# Autodesk Inventor assembly: ASM1001-001-005-320 - Controller Flash
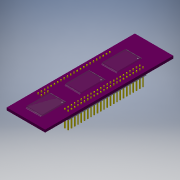
[picture p0: Inventor's stored thumbnail of the model, 180x180]
Saved by Autodesk Inventor 2019 (Build 230136000, 136)
## iProperties
Created: 2019-07-16
Part Number: ASM1001-001-005-320 - Controller Flash
Document SubType Name: Assembly
Designer: james
Author: james
## Documents named in this file (6)
- F:\JimsDesign\P1001-16bit-CPU\P1001-001 - 16bit CPU\P1001-001-005-320 - Controller Flash\ASM1001-001-005-320 - Controller Flash.iam
- F:\JimsDesign\P1001-16bit-CPU\P1001-001 - 16bit CPU\P1001-001-005-320 - Controller Flash\PRT1001-001-005-320 - Controller Flash.ipt
- F:\JimsDesign\P1001-16bit-CPU\P1001-001 - 16bit CPU\P1001-001-210 - CAD Library\UL_SST39VF1602704IEKE\2019-07-17_03-10-51\STEP\TSOP48_EKE_SST.ipt
- F:\JimsDesign\P1001-16bit-CPU\P1001-001 - 16bit CPU\P1001-001-210 - CAD Library\2X24Pins.iam
- F:\JimsDesign\P1001-16bit-CPU\P1001-001 - 16bit CPU\P1001-001-210 - CAD Library\1x20Pins.iam
- F:\JimsDesign\P1001-16bit-CPU\P1001-001 - 16bit CPU\P1001-001-210 - CAD Library\2x3pins.iam
## Components (7 placed, 5 different names)
1. PRT1001-001-005-320 - Controller Flash:1 — Mate:1, Mate:2, Mate:3, Mate:4, Mate:6, Flush:5, Flush:6, Mate:7, Flush:7, Flush:8
2. TSOP48_EKE_SST:1 — Mate:3, Flush:2
3. TSOP48_EKE_SST:2 — Mate:2, Flush:1, Flush:2
4. TSOP48_EKE_SST:3 — Mate:1, Mate:4, Flush:1
5. 2X24Pins:1 [sub-assembly] — Mate:7, Flush:7, Flush:8
6. 1x20Pins:1 [sub-assembly] — Mate:5, Flush:3, Flush:4, Mate:6, Flush:5
7. 2x3pins:1 [sub-assembly] — Mate:5, Flush:3, Flush:4, Flush:6
## Relationships (15: Flush 8, Mate 7)
- Mate:1: PRT1001-001-005-320 - Controller Flash:1 ↔ TSOP48_EKE_SST:3
- Mate:2: PRT1001-001-005-320 - Controller Flash:1 ↔ TSOP48_EKE_SST:2
- Mate:3: PRT1001-001-005-320 - Controller Flash:1 ↔ TSOP48_EKE_SST:1
- Mate:4 (10 mm): PRT1001-001-005-320 - Controller Flash:1 ↔ TSOP48_EKE_SST:3
- Flush:1: TSOP48_EKE_SST:2 ↔ TSOP48_EKE_SST:3
- Flush:2: TSOP48_EKE_SST:1 ↔ TSOP48_EKE_SST:2
- Mate:5: 1x20Pins:1 ↔ 2x3pins:1
- Flush:3: 1x20Pins:1 ↔ 2x3pins:1
- Flush:4: 1x20Pins:1 ↔ 2x3pins:1
- Mate:6: PRT1001-001-005-320 - Controller Flash:1 ↔ 1x20Pins:1
- Flush:5 (2 mm): PRT1001-001-005-320 - Controller Flash:1 ↔ 1x20Pins:1
- Flush:6 (20 mm): PRT1001-001-005-320 - Controller Flash:1 ↔ 2x3pins:1
- Mate:7: PRT1001-001-005-320 - Controller Flash:1 ↔ 2X24Pins:1
- Flush:7 (20 mm): PRT1001-001-005-320 - Controller Flash:1 ↔ 2X24Pins:1
- Flush:8 (2 mm): PRT1001-001-005-320 - Controller Flash:1 ↔ 2X24Pins:1
